# Autodesk Inventor assembly: Chessboard Top
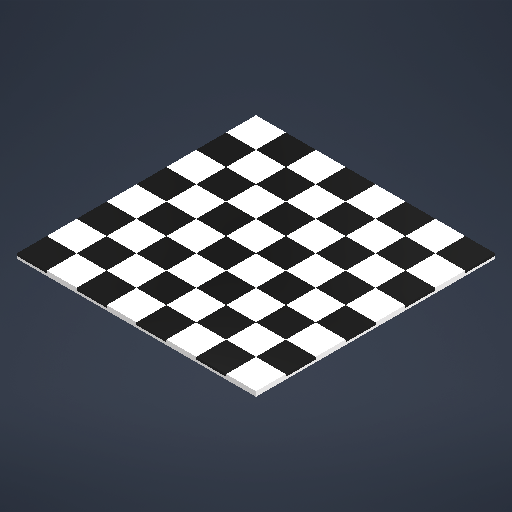
[picture p0: Inventor's stored thumbnail of the model, 512x512]
Saved by Autodesk Inventor 2026 (Build 300175000, 175)
## iProperties
Created: 2025-04-18
Part Number: Chessboard Top
Document SubType Name: Assembly
Designer: ckyiu
Author: ckyiu
## Documents named in this file (5)
- C:\Users\ckyiu\Documents\Projects\Chessboard-Design\Assemblies\Chessboard Top.iam
- C:\Users\ckyiu\Documents\Projects\Chessboard-Design\Parts\Square Holder.ipt
- C:\Users\ckyiu\Documents\Projects\Chessboard-Design\Parts\White Square.ipt
- C:\Users\ckyiu\Documents\Projects\Chessboard-Design\Parts\Black Square.ipt
- C:\Users\ckyiu\Documents\Projects\Chessboard-Design\Parts\Generic Neodynium Magnet 10mm diameter 2mm height.ipt
## Components (129 placed, 4 different names)
1. Square Holder:1 — Flush:1, Flush:2, Mate:1, Mate:2, Flush:3, Flush:4, Mate:3, Flush:5, Flush:6, Mate:4, Flush:7, Flush:8, Insert:1
2. White Square:1 — Flush:1, Flush:2, Mate:1
3. White Square:2
4. White Square:3
5. White Square:4
6. White Square:5
7. White Square:6
8. White Square:7
9. White Square:8
10. White Square:9
11. White Square:10
12. White Square:11
13. White Square:12
14. White Square:13
15. White Square:14
16. White Square:15
17. White Square:16
18. White Square:17 — Mate:2, Flush:3, Flush:4
19. White Square:18
20. White Square:19
21. White Square:20
22. White Square:21
23. White Square:22
24. White Square:23
25. White Square:24
26. White Square:25
27. White Square:26
28. White Square:27
29. White Square:28
30. White Square:29
31. White Square:30
32. White Square:31
33. White Square:32
34. Black Square:1 — Mate:3, Flush:5, Flush:6
35. Black Square:2
36. Black Square:3
37. Black Square:4
38. Black Square:5
39. Black Square:6
40. Black Square:7
41. Black Square:8
42. Black Square:9
43. Black Square:10
44. Black Square:11
45. Black Square:12
46. Black Square:13
47. Black Square:14
48. Black Square:15
49. Black Square:16
50. Black Square:17 — Mate:4, Flush:7, Flush:8
51. Black Square:18
52. Black Square:19
53. Black Square:20
54. Black Square:21
55. Black Square:22
56. Black Square:23
57. Black Square:24
58. Black Square:25
59. Black Square:26
60. Black Square:27
61. Black Square:28
62. Black Square:29
63. Black Square:30
64. Black Square:31
65. Black Square:32
66. Generic Neodynium Magnet 10mm diameter 2mm height:1 — Insert:1
67. Generic Neodynium Magnet 10mm diameter 2mm height:2
68. Generic Neodynium Magnet 10mm diameter 2mm height:3
69. Generic Neodynium Magnet 10mm diameter 2mm height:4
70. Generic Neodynium Magnet 10mm diameter 2mm height:5
71. Generic Neodynium Magnet 10mm diameter 2mm height:6
72. Generic Neodynium Magnet 10mm diameter 2mm height:7
73. Generic Neodynium Magnet 10mm diameter 2mm height:8
74. Generic Neodynium Magnet 10mm diameter 2mm height:9
75. Generic Neodynium Magnet 10mm diameter 2mm height:10
76. Generic Neodynium Magnet 10mm diameter 2mm height:11
77. Generic Neodynium Magnet 10mm diameter 2mm height:12
78. Generic Neodynium Magnet 10mm diameter 2mm height:13
79. Generic Neodynium Magnet 10mm diameter 2mm height:14
80. Generic Neodynium Magnet 10mm diameter 2mm height:15
81. Generic Neodynium Magnet 10mm diameter 2mm height:16
82. Generic Neodynium Magnet 10mm diameter 2mm height:17
83. Generic Neodynium Magnet 10mm diameter 2mm height:18
84. Generic Neodynium Magnet 10mm diameter 2mm height:19
85. Generic Neodynium Magnet 10mm diameter 2mm height:20
86. Generic Neodynium Magnet 10mm diameter 2mm height:21
87. Generic Neodynium Magnet 10mm diameter 2mm height:22
88. Generic Neodynium Magnet 10mm diameter 2mm height:23
89. Generic Neodynium Magnet 10mm diameter 2mm height:24
90. Generic Neodynium Magnet 10mm diameter 2mm height:25
91. Generic Neodynium Magnet 10mm diameter 2mm height:26
92. Generic Neodynium Magnet 10mm diameter 2mm height:27
93. Generic Neodynium Magnet 10mm diameter 2mm height:28
94. Generic Neodynium Magnet 10mm diameter 2mm height:29
95. Generic Neodynium Magnet 10mm diameter 2mm height:30
96. Generic Neodynium Magnet 10mm diameter 2mm height:31
97. Generic Neodynium Magnet 10mm diameter 2mm height:32
98. Generic Neodynium Magnet 10mm diameter 2mm height:33
99. Generic Neodynium Magnet 10mm diameter 2mm height:34
100. Generic Neodynium Magnet 10mm diameter 2mm height:35
101. Generic Neodynium Magnet 10mm diameter 2mm height:36
102. Generic Neodynium Magnet 10mm diameter 2mm height:37
103. Generic Neodynium Magnet 10mm diameter 2mm height:38
104. Generic Neodynium Magnet 10mm diameter 2mm height:39
105. Generic Neodynium Magnet 10mm diameter 2mm height:40
106. Generic Neodynium Magnet 10mm diameter 2mm height:41
107. Generic Neodynium Magnet 10mm diameter 2mm height:42
108. Generic Neodynium Magnet 10mm diameter 2mm height:43
109. Generic Neodynium Magnet 10mm diameter 2mm height:44
110. Generic Neodynium Magnet 10mm diameter 2mm height:45
111. Generic Neodynium Magnet 10mm diameter 2mm height:46
112. Generic Neodynium Magnet 10mm diameter 2mm height:47
113. Generic Neodynium Magnet 10mm diameter 2mm height:48
114. Generic Neodynium Magnet 10mm diameter 2mm height:49
115. Generic Neodynium Magnet 10mm diameter 2mm height:50
116. Generic Neodynium Magnet 10mm diameter 2mm height:51
117. Generic Neodynium Magnet 10mm diameter 2mm height:52
118. Generic Neodynium Magnet 10mm diameter 2mm height:53
119. Generic Neodynium Magnet 10mm diameter 2mm height:54
120. Generic Neodynium Magnet 10mm diameter 2mm height:55
121. Generic Neodynium Magnet 10mm diameter 2mm height:56
122. Generic Neodynium Magnet 10mm diameter 2mm height:57
123. Generic Neodynium Magnet 10mm diameter 2mm height:58
124. Generic Neodynium Magnet 10mm diameter 2mm height:59
125. Generic Neodynium Magnet 10mm diameter 2mm height:60
126. Generic Neodynium Magnet 10mm diameter 2mm height:61
127. Generic Neodynium Magnet 10mm diameter 2mm height:62
128. Generic Neodynium Magnet 10mm diameter 2mm height:63
129. Generic Neodynium Magnet 10mm diameter 2mm height:64
## Component patterns: (16 elements, first: White Square:1), (16 elements, first: White Square:17), (16 elements, first: Black Square:1), (16 elements, first: Black Square:17), (64 elements, first: Generic Neodynium Magnet 10mm diameter 2mm height:1)
## Relationships (13: Flush 8, Mate 4, Insert 1)
- Flush:1: Square Holder:1 ↔ White Square:1
- Flush:2: Square Holder:1 ↔ White Square:1
- Mate:1: Square Holder:1 ↔ White Square:1
- Mate:2: Square Holder:1 ↔ White Square:17
- Flush:3: Square Holder:1 ↔ White Square:17
- Flush:4: Square Holder:1 ↔ White Square:17
- Mate:3: Square Holder:1 ↔ Black Square:1
- Flush:5: Square Holder:1 ↔ Black Square:1
- Flush:6: Square Holder:1 ↔ Black Square:1
- Mate:4: Square Holder:1 ↔ Black Square:17
- Flush:7: Square Holder:1 ↔ Black Square:17
- Flush:8: Square Holder:1 ↔ Black Square:17
- Insert:1: Square Holder:1 ↔ Generic Neodynium Magnet 10mm diameter 2mm height:1
